# Autodesk Inventor assembly: omni_frame
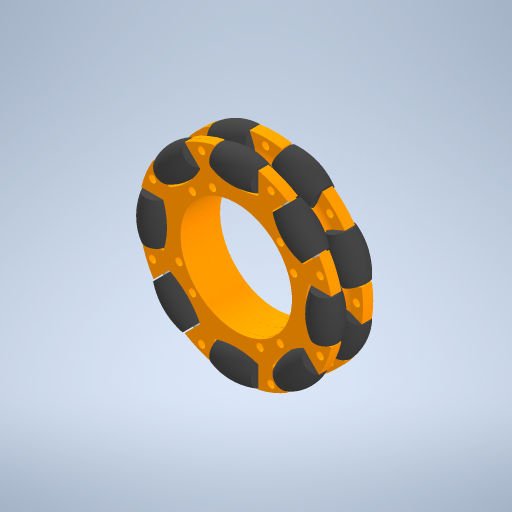
[picture p0: Inventor's stored thumbnail of the model, 512x512]
Saved by Autodesk Inventor 2024.1 (Build 281209000, 209)
## iProperties
Created: 2024-11-27
Part Number: omni_frame
Document SubType Name: Assembly
Designer: hibik
Author: hibik
## Documents named in this file (2)
- C:\Users\hibik\Documents\Robomech\RESCUE\ORCA\hard\omni_wheel\omni_wheel.iam
- C:\Users\hibik\Documents\Robomech\RESCUE\ORCA\hard\omni_wheel\omni_harf_frame.iam
## Components (2 placed, 1 different names)
1. omni_harf_frame:1 [sub-assembly] — 挿入:1, 挿入:2
2. omni_harf_frame:2 [sub-assembly] — 挿入:1, 挿入:2
## Relationships (2: Insert 2)
- 挿入:1 [Insert]: omni_harf_frame:1 ↔ omni_harf_frame:2
- 挿入:2 [Insert]: omni_harf_frame:1 ↔ omni_harf_frame:2
